# Autodesk Inventor assembly: crank_motor_mount
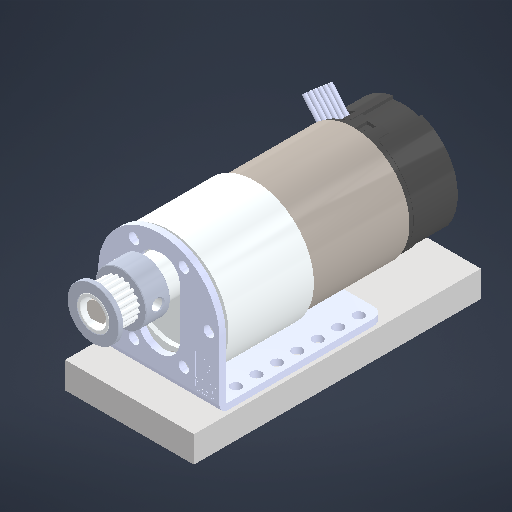
[picture p0: Inventor's stored thumbnail of the model, 512x512]
Saved by Autodesk Inventor 2026 (Build 300175050, 175E)
## iProperties
Created: 2025-11-11
Part Number: crank_motor_mount
Document SubType Name: Assembly
Designer: habbo
Author: habbo
## Documents named in this file (5)
- C:\Users\habbo\OneDrive\Documents\GitHub\Tesis_Mecanismo\CAD\Piezas Variadas\crank_motor_mount.iam
- C:\Users\habbo\OneDrive\Documents\GitHub\Tesis_Mecanismo\CAD\Piezas Variadas\37d-gearmotor-100-131-encoder.ipt
- C:\Users\habbo\OneDrive\Documents\GitHub\Tesis_Mecanismo\CAD\Piezas Variadas\pololu-stamped-aluminum-l-bracket-for-37d-mm-metal-gearmotors.ipt
- C:\Users\habbo\OneDrive\Documents\GitHub\Tesis_Mecanismo\CAD\Piezas Variadas\motor_bracket_base.ipt
- C:\Users\habbo\OneDrive\Documents\GitHub\Tesis_Mecanismo\CAD\Piezas Variadas\GT2 Timing Pulley, Configurable, 20T W6 B8.ipt
## Components (4 placed, 4 different names)
1. pololu-stamped-aluminum-l-bracket-for-37d-mm-metal-gearmotors:1 — Mate:1, Mate:2, Flush:2, Mate:6, Flush:3
2. 37d-gearmotor-100-131-encoder:1 — Mate:1, Mate:2, Mate:4, Mate:5
3. motor_bracket_base:1 — Flush:2, Mate:6, Flush:3
4. GT2 Timing Pulley, Configurable, 20T W6 B8:1 — Mate:4, Mate:5
## Relationships (7: Mate 5, Flush 2)
- Mate:1: pololu-stamped-aluminum-l-bracket-for-37d-mm-metal-gearmotors:1 ↔ 37d-gearmotor-100-131-encoder:1
- Mate:2: pololu-stamped-aluminum-l-bracket-for-37d-mm-metal-gearmotors:1 ↔ 37d-gearmotor-100-131-encoder:1
- Flush:2 (1.204 mm): pololu-stamped-aluminum-l-bracket-for-37d-mm-metal-gearmotors:1 ↔ motor_bracket_base:1
- Mate:4: 37d-gearmotor-100-131-encoder:1 ↔ GT2 Timing Pulley, Configurable, 20T W6 B8:1
- Mate:5 (1 mm): 37d-gearmotor-100-131-encoder:1 ↔ GT2 Timing Pulley, Configurable, 20T W6 B8:1
- Mate:6: pololu-stamped-aluminum-l-bracket-for-37d-mm-metal-gearmotors:1 ↔ motor_bracket_base:1
- Flush:3 (9.1 mm): pololu-stamped-aluminum-l-bracket-for-37d-mm-metal-gearmotors:1 ↔ motor_bracket_base:1
